# Autodesk Inventor assembly: Middle Rod Assembly
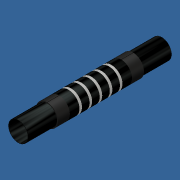
[picture p0: Inventor's stored thumbnail of the model, 180x180]
Saved by Autodesk Inventor 2018 (Build 220112000, 112)
## iProperties
Created: 2018-02-27
Part Number: Middle Rod Assembly
Document SubType Name: Assembly
Designer: 232963
Author: 232963
## Documents named in this file (4)
- D:\Cole\Documents\GitHub\SchoolCAD\ReverseEngineering\Middle Rod Assembly.iam
- D:\Cole\Documents\GitHub\SchoolCAD\ReverseEngineering\Middle Rod.ipt
- D:\Cole\Documents\GitHub\SchoolCAD\ReverseEngineering\MIddle Rod Cover.ipt
- D:\Cole\Documents\GitHub\SchoolCAD\ReverseEngineering\Buffer Piece.ipt
## Components (4 placed, 3 different names)
1. Middle Rod:1 — Insert:1
2. MIddle Rod Cover:1 — Insert:1, Insert:2, Insert:3
3. Buffer Piece:1 — Insert:3
4. Buffer Piece:2 — Insert:2
## Relationships (3: Insert 3)
- Insert:1 (64.77 mm): Middle Rod:1 ↔ MIddle Rod Cover:1
- Insert:2: MIddle Rod Cover:1 ↔ Buffer Piece:2
- Insert:3: MIddle Rod Cover:1 ↔ Buffer Piece:1
